# Autodesk Inventor assembly: Full Pull Drawer
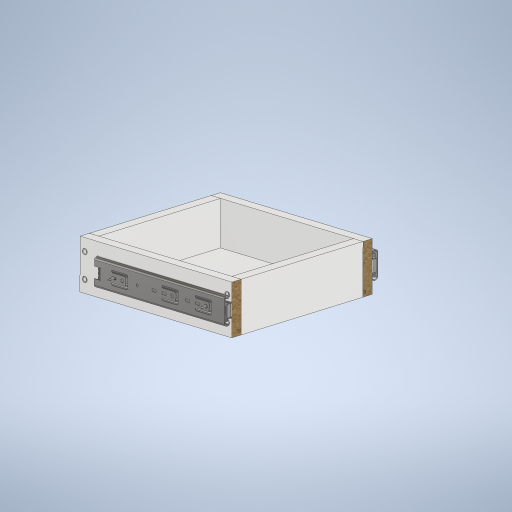
[picture p0: Inventor's stored thumbnail of the model, 512x512]
Saved by Autodesk Inventor 2024 (Build 280153000, 153)
## iProperties
Category: Drawer
RuleStatus: InUse
Created: 2013-11-19
Part Number: Full Pull Drawer
Document SubType Name: Assembly
Designer: SauliusD
Description: Full Pull Drawer
AfterAnyUserParamChange0: Drawer Configuration
Author: SauliusD
## Documents named in this file (10)
- C:\W4INV 2024 Design\iBOX LIBRARY\Drawers\Full Pull Drawer\Full Pull Drawer.iam
- C:\W4INV 2024 Design\iBOX LIBRARY\Drawers\Full Pull Drawer\Parts\DR Left.ipt
- C:\W4INV 2024 Design\iBOX LIBRARY\Drawers\Full Pull Drawer\Parts\DR Right.ipt
- C:\W4INV 2024 Design\iBOX LIBRARY\Drawers\Full Pull Drawer\Parts\DR Back.ipt
- C:\W4INV 2024 Design\iBOX LIBRARY\Drawers\Full Pull Drawer\Parts\DR Front.ipt
- C:\W4INV 2024 Design\iBOX LIBRARY\Drawers\Full Pull Drawer\Parts\DR Bottom.ipt
- C:\W4INV 2024 Design\iBOX LIBRARY\Drawers\Full Pull Drawer\Parts\Full Extension Ball bearing Slide.iam
- C:\W4INV 2024 Design\iBOX LIBRARY\Drawers\Full Pull Drawer\Full Pull Drawer.ipt
- C:\W4INV 2024 Design\_LIBRARY\Fixed joints\Confirmat\CONFIRMAT\Confirmat L50 NB T18 PB T 18.ipt
- C:\W4INV 2024 Design\LIBRARY\Fixed joints\Confirmat\CONFIRMAT.ipt
## Components (16 placed, 15 different names)
1. @Skeleton — Flush:16, Flush:17, Flush:18
2. Full Extension Ball bearing Slide:1 [sub-assembly] — Flush:2, Flush:3, Flush:4, Flush:5
3. DR Left:1 — Mate:1, Flush:1, Nestled Board Plane:1, Nestled Board Plane:3, Nestled Board Plane:5, Nestled Board Plane:7
4. DR Right:1 — Nestled Board Plane:2, Nestled Board Plane:4, Nestled Board Plane:6, Nestled Board Plane:8
5. DR Back:1 — Second Axis Plane:1, Second Axis Plane:2, Second Axis Plane:3, Second Axis Plane:4
6. DR Front:1 — Flush:6, Flush:7, Second Axis Plane:5, Second Axis Plane:6, Second Axis Plane:7, Second Axis Plane:8
7. DR Bottom:1
8. Full Extension Ball bearing Slide:2 [sub-assembly] — Mate:1, Flush:1, Flush:2
9. Confirmat 1 — Second Axis Plane:1, Axis Plane:1, Nestled Board Plane:1
10. Confirmat 2 — Second Axis Plane:2, Axis Plane:2, Nestled Board Plane:2
11. Confirmat 3 — Second Axis Plane:3, Axis Plane:3, Nestled Board Plane:3
12. Confirmat 4 — Second Axis Plane:4, Axis Plane:4, Nestled Board Plane:4
13. Confirmat 5 — Second Axis Plane:5, Axis Plane:5, Nestled Board Plane:5
14. Confirmat 6 — Second Axis Plane:6, Axis Plane:6, Nestled Board Plane:6
15. Confirmat 7 — Second Axis Plane:7, Axis Plane:7, Nestled Board Plane:7
16. Confirmat 8 — Second Axis Plane:8, Axis Plane:8, Nestled Board Plane:8
## Relationships (35: Flush 18, Mate 17)
- Mate:1: DR Left:1 ↔ Full Extension Ball bearing Slide:2
- Flush:1: DR Left:1 ↔ Full Extension Ball bearing Slide:2
- Flush:2: Full Extension Ball bearing Slide:1 ↔ Full Extension Ball bearing Slide:2
- Flush:3: Full Extension Ball bearing Slide:1
- Flush:4: Full Extension Ball bearing Slide:1
- Flush:5: Full Extension Ball bearing Slide:1
- Flush:6 (-20 mm): DR Front:1
- Flush:7 (-20 mm): DR Front:1
- Flush:16: @Skeleton
- Flush:17: @Skeleton
- Flush:18: @Skeleton
- Second Axis Plane:1 [Mate]: DR Back:1 ↔ Confirmat 1
- Axis Plane:1 [Mate]: Confirmat 1
- Nestled Board Plane:1 [Flush]: DR Left:1 ↔ Confirmat 1
- Second Axis Plane:2 [Mate]: DR Back:1 ↔ Confirmat 2
- Axis Plane:2 [Mate]: Confirmat 2
- Nestled Board Plane:2 [Flush]: DR Right:1 ↔ Confirmat 2
- Second Axis Plane:3 [Mate]: DR Back:1 ↔ Confirmat 3
- Axis Plane:3 [Mate]: Confirmat 3
- Nestled Board Plane:3 [Flush]: DR Left:1 ↔ Confirmat 3
- Second Axis Plane:4 [Mate]: DR Back:1 ↔ Confirmat 4
- Axis Plane:4 [Mate]: Confirmat 4
- Nestled Board Plane:4 [Flush]: DR Right:1 ↔ Confirmat 4
- Second Axis Plane:5 [Mate]: DR Front:1 ↔ Confirmat 5
- Axis Plane:5 [Mate]: Confirmat 5
- Nestled Board Plane:5 [Flush]: DR Left:1 ↔ Confirmat 5
- Second Axis Plane:6 [Mate]: DR Front:1 ↔ Confirmat 6
- Axis Plane:6 [Mate]: Confirmat 6
- Nestled Board Plane:6 [Flush]: DR Right:1 ↔ Confirmat 6
- Second Axis Plane:7 [Mate]: DR Front:1 ↔ Confirmat 7
- Axis Plane:7 [Mate]: Confirmat 7
- Nestled Board Plane:7 [Flush]: DR Left:1 ↔ Confirmat 7
- Second Axis Plane:8 [Mate]: DR Front:1 ↔ Confirmat 8
- Axis Plane:8 [Mate]: Confirmat 8
- Nestled Board Plane:8 [Flush]: DR Right:1 ↔ Confirmat 8
## Named parameters: ConfirmatOffset = -20 mm, Inlet_Drawer = 0 mm, Rear_Space = 20 mm, Drawer_H = 100 mm, Inlet = 0 mm, Board_T = 18 mm, Distance_from_bottom = 0 mm
